# Autodesk Inventor assembly: smietnik1_zlozenie
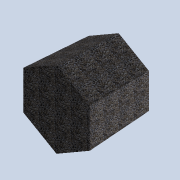
[picture p0: Inventor's stored thumbnail of the model, 180x180]
Saved by Autodesk Inventor 2021 (Build 250183000, 183)
## iProperties
Created: 2025-11-29
Part Number: smietnik1_zlozenie
Document SubType Name: Assembly
Designer: huber
Author: huber
## Documents named in this file (6)
- C:\Users\huber\OneDrive\Pulpit\hackaton BHL\BHL 2025\smietnik1_zlozenie.iam
- C:\Users\huber\OneDrive\Pulpit\hackaton BHL\BHL 2025\smietnik1.ipt
- C:\Users\huber\OneDrive\Pulpit\hackaton BHL\BHL 2025\smietnik1_srodek.ipt
- C:\Users\huber\OneDrive\Pulpit\hackaton BHL\BHL 2025\zlozenie_kompetne_WIZUAL.iam
- C:\Users\huber\OneDrive\Dokumenty\Inventor\Content Center Files\R2021\en-US\ISO 4016\ISO 4016 - M8 x 40.ipt
- C:\Users\huber\Downloads\Solar Panel.ipt
## Components (6 placed, 5 different names)
1. smietnik1:1 — Insert:1, Mate:2, Mate:3
2. smietnik1_srodek:1 — Insert:1
3. zlozenie_kompetne_WIZUAL:1 [sub-assembly] — Mate:3, Flush:1, Insert:2, Insert:3, Flush:2, Mate:4, Flush:3
4. ISO 4016 M8 x 40:1 — Insert:2
5. ISO 4016 M8 x 40:2 — Insert:3
6. Solar Panel:1 — Flush:2, Mate:4, Flush:3
## Relationships (10: Insert 3, Mate 3, Flush 3, Angle 1)
- Insert:1: smietnik1:1 ↔ smietnik1_srodek:1
- Mate:2: smietnik1:1
- Angle:1 (180 deg)
- Mate:3: smietnik1:1 ↔ zlozenie_kompetne_WIZUAL:1
- Flush:1: zlozenie_kompetne_WIZUAL:1
- Insert:2: zlozenie_kompetne_WIZUAL:1 ↔ ISO 4016 M8 x 40:1
- Insert:3: zlozenie_kompetne_WIZUAL:1 ↔ ISO 4016 M8 x 40:2
- Flush:2 (2.223 mm): zlozenie_kompetne_WIZUAL:1 ↔ Solar Panel:1
- Mate:4: zlozenie_kompetne_WIZUAL:1 ↔ Solar Panel:1
- Flush:3 (4.375 mm): zlozenie_kompetne_WIZUAL:1 ↔ Solar Panel:1
